# Autodesk Inventor assembly: Short Arm
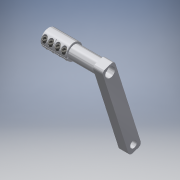
[picture p0: Inventor's stored thumbnail of the model, 180x180]
Saved by Autodesk Inventor 2016 (Build 200138000, 138)
## iProperties
Created: 2015-06-08
Part Number: Short Arm
Document SubType Name: Assembly
Designer: Dennis
Author: Dennis
## Documents named in this file (4)
- C:\Users\Dennis\Dropbox\NI Work\NI Slider Crank\Assemblies\Short Arm.iam
- C:\Users\Dennis\Dropbox\NI Work\NI Slider Crank\Parts\0.250 - 0.250 Coupler - 61005K311.ipt
- C:\Users\Dennis\Dropbox\NI Work\NI Slider Crank\Parts\Pin.ipt
- C:\Users\Dennis\Dropbox\NI Work\NI Slider Crank\Parts\Arm Short.ipt
## Components (3 placed, 3 different names)
1. 0.250 - 0.250 Coupler - 61005K311:1 — Mate:1, Flush:1, Angle:1
2. Pin:1 — Mate:1, Flush:1, Mate:2, Mate:3
3. Arm Short:1 — Mate:2, Mate:3, Angle:1
## Relationships (5: Mate 3, Flush 1, Angle 1)
- Mate:1: 0.250 - 0.250 Coupler - 61005K311:1 ↔ Pin:1
- Flush:1: 0.250 - 0.250 Coupler - 61005K311:1 ↔ Pin:1
- Mate:2: Pin:1 ↔ Arm Short:1
- Mate:3: Pin:1 ↔ Arm Short:1
- Angle:1 (0 deg): 0.250 - 0.250 Coupler - 61005K311:1 ↔ Arm Short:1
